# Autodesk Inventor assembly: sanfrancisco
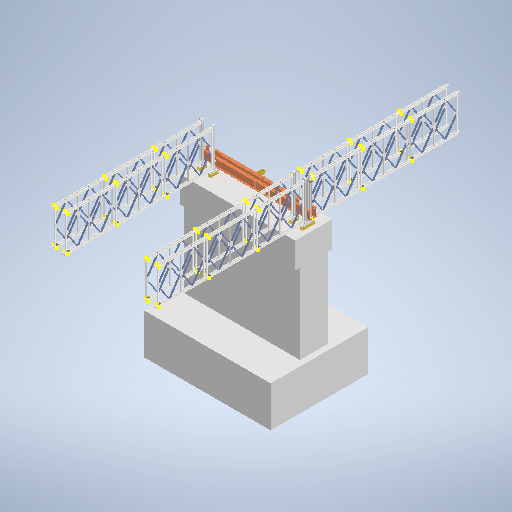
[picture p0: Inventor's stored thumbnail of the model, 512x512]
Saved by Autodesk Inventor 2025 (Build 290162000, 162)
## iProperties
Created: 2024-09-24
Part Number: sanfrancisco
Document SubType Name: Assembly
Designer: jfelix
Author: jfelix
## Documents named in this file (8)
- D:\provias\2024\MODELOS INVENTOR\HARZONE CB200A\sanfrancisco.iam
- D:\provias\2024\MODELOS INVENTOR\Pilar san francisco.ipt
- D:\provias\2024\MODELOS INVENTOR\HARZONE CB200A\panel standar.iam
- D:\provias\2024\MODELOS INVENTOR\HARZONE CB200A\CB740A.ipt
- D:\provias\2024\MODELOS INVENTOR\HARZONE CB200A\CB370A.ipt
- D:\provias\2024\MODELOS INVENTOR\HARZONE CB200A\CB700A.ipt
- D:\provias\2024\MODELOS INVENTOR\HARZONE CB200A\VIGA TRANSVERSAL.ipt
- D:\provias\2024\MODELOS INVENTOR\HARZONE CB200A\CB710A.ipt
## Components (38 placed, 7 different names)
1. Pilar san francisco:2 — Coincidencia:1, Coincidencia:2, Coincidencia:3, Coincidencia:4, Ángulo:5
2. CB740A:2 — Coincidencia:4, Nivelación:1, Nivelación:2, Coincidencia:13, Tangente:2, Tangente:3, Nivelación:7
3. VIGA TRANSVERSAL:1 — Coincidencia:18, Ángulo:6, Coincidencia:19, Nivelación:8
4. CB710A:1 — Coincidencia:15, Coincidencia:16, Coincidencia:17
5. CB370A:2 — Coincidencia:13, Tangente:2, Tangente:3, Nivelación:7, Coincidencia:17, Ángulo:6
6. VIGA TRANSVERSAL:2 — Nivelación:8, Coincidencia:20, Coincidencia:21
7. CB740A:6
8. CB740A:7
9. panel standar:1 [sub-assembly] — Nivelación:5, Coincidencia:15, Coincidencia:16, Ángulo:5, Coincidencia:20, Coincidencia:21
10. panel standar:8 [sub-assembly]
11. panel standar:9 [sub-assembly]
12. panel standar:10 [sub-assembly]
13. panel standar:11 [sub-assembly]
14. panel standar:12 [sub-assembly]
15. panel standar:2 [sub-assembly] — Coincidencia:9, Nivelación:5, Coincidencia:14
16. panel standar:3 [sub-assembly]
17. panel standar:4 [sub-assembly]
18. panel standar:5 [sub-assembly]
19. panel standar:6 [sub-assembly]
20. panel standar:7 [sub-assembly]
21. panel standar:13 [sub-assembly]
22. panel standar:14 [sub-assembly]
23. panel standar:15 [sub-assembly]
24. panel standar:16 [sub-assembly]
25. panel standar:17 [sub-assembly]
26. panel standar:18 [sub-assembly]
27. CB740A:1 — Coincidencia:1, Coincidencia:2, Coincidencia:3, Nivelación:1, Nivelación:2, Ángulo:2, Ángulo:3, Tangente:1, Ángulo:4, Coincidencia:12, Nivelación:6
28. CB370A:1 — Tangente:1, Ángulo:4, Coincidencia:11, Coincidencia:12, Nivelación:6
29. CB700A:1 — Ángulo:2, Ángulo:3, Coincidencia:9, Coincidencia:11, Coincidencia:14, Coincidencia:18, Coincidencia:19
30. CB740A:3
31. CB370A:3
32. CB700A:2
33. CB740A:4
34. CB370A:4
35. CB700A:3
36. CB740A:5
37. CB370A:5
38. CB700A:4
## Component patterns: (6 elements, first: panel standar:1), (2 elements), (2 elements), (6 elements, first: panel standar:2), Patrón de componentes 1:2 (6 elements), (2 elements, first: CB740A:1 + CB370A:1 + CB700A:1), Patrón de componentes 4:2 (2 elements)
## Relationships (30: Mate 16, Flush 6, Angle 5, Tangent 3)
- Coincidencia:1 [Mate]: Pilar san francisco:2 ↔ CB740A:1
- Coincidencia:2 [Mate]: Pilar san francisco:2 ↔ CB740A:1
- Coincidencia:3 [Mate]: Pilar san francisco:2 ↔ CB740A:1
- Coincidencia:4 [Mate]: Pilar san francisco:2 ↔ CB740A:2
- Nivelación:1 [Flush]: CB740A:2 ↔ CB740A:1
- Nivelación:2 [Flush]: CB740A:2 ↔ CB740A:1
- Ángulo:2 [Angle] (0 deg): CB740A:1 ↔ CB700A:1
- Ángulo:3 [Angle] (0 deg): CB740A:1 ↔ CB700A:1
- Tangente:1: CB740A:1 ↔ CB370A:1
- Ángulo:4 [Angle] (0 deg): CB740A:1 ↔ CB370A:1
- Coincidencia:9 [Mate]: panel standar:2 ↔ CB700A:1
- Nivelación:5 [Flush]: panel standar:1 ↔ panel standar:2
- Coincidencia:11 [Mate]: CB370A:1 ↔ CB700A:1
- Coincidencia:12 [Mate]: CB740A:1 ↔ CB370A:1
- Nivelación:6 [Flush] (-15 mm): CB740A:1 ↔ CB370A:1
- Coincidencia:13 [Mate]: CB740A:2 ↔ CB370A:2
- Tangente:2: CB740A:2 ↔ CB370A:2
- Tangente:3: CB740A:2 ↔ CB370A:2
- Nivelación:7 [Flush] (-15 mm): CB740A:2 ↔ CB370A:2
- Coincidencia:14 [Mate]: panel standar:2 ↔ CB700A:1
- Coincidencia:15 [Mate]: CB710A:1 ↔ panel standar:1
- Coincidencia:16 [Mate]: CB710A:1 ↔ panel standar:1
- Coincidencia:17 [Mate]: CB710A:1 ↔ CB370A:2
- Ángulo:5 [Angle] (0 deg): Pilar san francisco:2 ↔ panel standar:1
- Coincidencia:18 [Mate]: VIGA TRANSVERSAL:1 ↔ CB700A:1
- Ángulo:6 [Angle] (0 deg): VIGA TRANSVERSAL:1 ↔ CB370A:2
- Coincidencia:19 [Mate]: VIGA TRANSVERSAL:1 ↔ CB700A:1
- Nivelación:8 [Flush]: VIGA TRANSVERSAL:1 ↔ VIGA TRANSVERSAL:2
- Coincidencia:20 [Mate]: VIGA TRANSVERSAL:2 ↔ panel standar:1
- Coincidencia:21 [Mate]: VIGA TRANSVERSAL:2 ↔ panel standar:1
